# Autodesk Inventor assembly: ChassisDes1
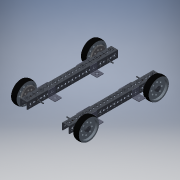
[picture p0: Inventor's stored thumbnail of the model, 180x180]
Saved by Autodesk Inventor 2016 (Build 200138000, 138)
## iProperties
Created: 2015-08-30
Part Number: ChassisDes1
Document SubType Name: Assembly
Designer: Tim
Author: Tim
## Documents named in this file (3)
- C:\Users\Tim\Documents\GitHub\phi_robotics\3d-models\FTC_Tetrix_KOP_Block_Party\ChassisDes1.iam
- C:\Users\Tim\Documents\GitHub\phi_robotics\3d-models\FTC_Tetrix_KOP_Block_Party\RollingSquareC1.iam
- C:\Users\Tim\Documents\GitHub\phi_robotics\3d-models\FTC_Tetrix_KOP_Block_Party\Tetrix_Kit_FTC\Autodesk Inventor Files\tetrix_corner_bracket.ipt
## Components (10 placed, 2 different names)
1. tetrix_corner_bracket:1 — Rigid:2
2. tetrix_corner_bracket:2 — Rigid:1
3. RollingSquareC1:1 [sub-assembly] — Rigid:1, Rigid:2, Rigid:4, Rigid:6
4. tetrix_corner_bracket:3 — Rigid:4
5. tetrix_corner_bracket:4 — Rigid:6
6. RollingSquareC1:2 [sub-assembly]
7. tetrix_corner_bracket:5
8. tetrix_corner_bracket:6
9. tetrix_corner_bracket:7
10. tetrix_corner_bracket:8
## Relationships (8: WeldJoint 8)
- Rigid:1 [WeldJoint]: tetrix_corner_bracket:2 ↔ RollingSquareC1:1
- Rigid:2 [WeldJoint]: tetrix_corner_bracket:1 ↔ RollingSquareC1:1
- Rigid:4 [WeldJoint]: RollingSquareC1:1 ↔ tetrix_corner_bracket:3
- Rigid:6 [WeldJoint]: RollingSquareC1:1 ↔ tetrix_corner_bracket:4
- [WeldJoint]: RollingSquareC1:2 ↔ tetrix_corner_bracket:6
- [WeldJoint]: RollingSquareC1:2 ↔ tetrix_corner_bracket:5
- [WeldJoint]: RollingSquareC1:2 ↔ tetrix_corner_bracket:7
- [WeldJoint]: RollingSquareC1:2 ↔ tetrix_corner_bracket:8
## Named parameters: d9_d4 = 0 mm, d10_d8 = 0 mm, d11_d0 = 0 mm, d12_d1 = 0 mm
